# Autodesk Inventor assembly: LINK1
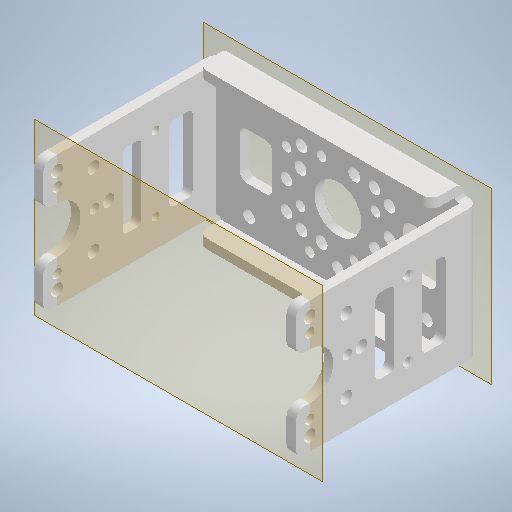
[picture p0: Inventor's stored thumbnail of the model, 512x512]
Saved by Autodesk Inventor 2026.1 (Build 301233020, 233B)
## iProperties
Created: 2025-10-15
Part Number: LINK1
Document SubType Name: Assembly
Designer: wlgns
Author: wlgns
## Documents named in this file (2)
- C:\Users\wlgns\Desktop\project\ARA Project\ARA_CAD_model\ARA_v2\LINK1.iam
- C:\Users\wlgns\Desktop\project\ARA Project\ARA_CAD_model\ARA_v2\FR08-H101.ipt
## Components (1 placed, 1 different names)
1. FR08-H101:1 — 메이트:1, 메이트:2, 메이트:3, 플러쉬:1
## Relationships (4: Mate 3, Flush 1)
- 메이트:1 [Mate]: FR08-H101:1
- 메이트:2 [Mate]: FR08-H101:1
- 메이트:3 [Mate]: FR08-H101:1
- 플러쉬:1 [Flush] (-3 mm): FR08-H101:1
